# Autodesk Inventor assembly: Bed Frame
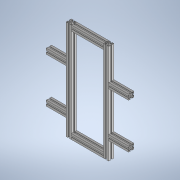
[picture p0: Inventor's stored thumbnail of the model, 180x180]
Saved by Autodesk Inventor 2022 (Build 260153000, 153)
## iProperties
Created: 2022-03-12
Part Number: Bed Frame
Document SubType Name: Assembly
Designer: Nick
Author: Nick
## Documents named in this file (4)
- Y:\Projects\Bibble0\SubAsm\Bed Frame.iam
- Y:\Projects\Bibble0\2020 Extrusions\Bed\2020 Bed Y.ipt
- Y:\Projects\Bibble0\2020 Extrusions\Bed\2020 Bed X.ipt
- Y:\Projects\Bibble0\2020 Extrusions\Bed\2020 Bed X - 75mm.ipt
## Components (8 placed, 3 different names)
1. 2020 Bed Y:1
2. 2020 Bed Y:2
3. 2020 Bed X:1
4. 2020 Bed X:2
5. 2020 Bed X - 75mm:1
6. 2020 Bed X - 75mm:2
7. 2020 Bed X - 75mm:3
8. 2020 Bed X - 75mm:4
## Relationships (17: Flush 10, Mate 7)
- [Flush]: 2020 Bed Y:1 ↔ 2020 Bed Y:2
- [Mate]: 2020 Bed Y:1 ↔ 2020 Bed X:1
- [Mate]: 2020 Bed Y:1 ↔ 2020 Bed X:2
- [Flush]: 2020 Bed Y:1 ↔ 2020 Bed X:2
- [Flush]: 2020 Bed Y:1 ↔ 2020 Bed X:2
- [Mate]: 2020 Bed Y:1 ↔ 2020 Bed X - 75mm:1
- [Flush]: 2020 Bed Y:1 ↔ 2020 Bed X - 75mm:1
- [Mate]: 2020 Bed Y:2 ↔ 2020 Bed X - 75mm:4
- [Flush]: 2020 Bed Y:2 ↔ 2020 Bed X - 75mm:4
- [Mate]: 2020 Bed Y:2 ↔ 2020 Bed X - 75mm:3
- [Flush]: 2020 Bed Y:2 ↔ 2020 Bed X - 75mm:3
- [Mate]: 2020 Bed Y:1 ↔ 2020 Bed X - 75mm:2
- [Flush]: 2020 Bed Y:1 ↔ 2020 Bed X - 75mm:2
- [Flush]: 2020 Bed Y:1 ↔ 2020 Bed X:1
- [Flush]: 2020 Bed Y:1 ↔ 2020 Bed X:1
- [Mate]: 2020 Bed Y:2 ↔ 2020 Bed X:1
- [Flush]: 2020 Bed Y:2 ↔ 2020 Bed X:1
